# Autodesk Inventor assembly: sp16-2p connector female
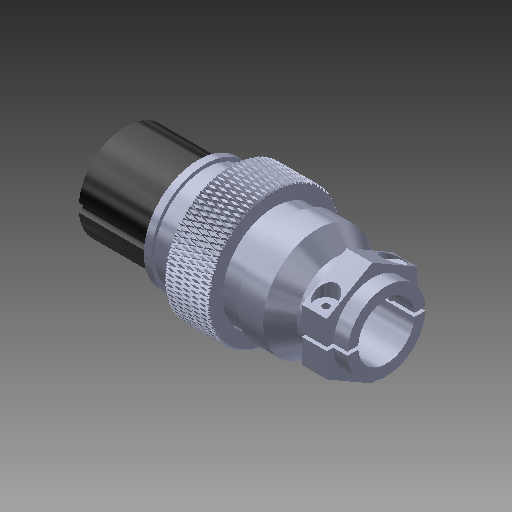
[picture p0: Inventor's stored thumbnail of the model, 512x512]
Saved by Autodesk Inventor 2018 (Build 220112000, 112)
## iProperties
Created: 2019-04-03
Part Number: sp16-2p connector female
Document SubType Name: Assembly
Designer: ZEUSLAP
Author: ZEUSLAP
## Documents named in this file (4)
- C:\Users\ZEUSLAP\YandexDisk\Inventor\solar_harvester_145x145\parts\sp16 waterproof connector\sp16-2p connector female.iam
- C:\Users\ZEUSLAP\YandexDisk\Inventor\solar_harvester_145x145\parts\sp16 waterproof connector\parts\2 pin body female.ipt
- C:\Users\ZEUSLAP\YandexDisk\Inventor\solar_harvester_145x145\parts\sp16 waterproof connector\parts\female_connector_shell.ipt
- C:\Users\ZEUSLAP\YandexDisk\Inventor\solar_harvester_145x145\parts\sp16 waterproof connector\parts\female_connector_ring.ipt
## Components (3 placed, 3 different names)
1. 2 pin body female:1 — Rotational:1
2. female_connector_shell:1 — Rotational:1, Mate:1, Mate:2
3. female_connector_ring:1 — Mate:1, Mate:2
## Relationships (3: Mate 2, RevoluteJoint 1)
- Rotational:1 [RevoluteJoint]: 2 pin body female:1 ↔ female_connector_shell:1
- Mate:1: female_connector_shell:1 ↔ female_connector_ring:1
- Mate:2 (3.5 mm): female_connector_shell:1 ↔ female_connector_ring:1
